# Autodesk Inventor assembly: BaseAssemblies
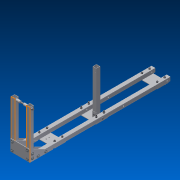
[picture p0: Inventor's stored thumbnail of the model, 180x180]
Saved by Autodesk Inventor 2013 (Build 170138000, 138)
## iProperties
Created: 2013-07-13
Part Number: BaseAssemblies
Document SubType Name: Assembly
Designer: orange
Mass: 2338.35 g
Surface Area: 7297.78 cm^2
Volume: 712.492 cm^3
Density: 3.28194 g/cm^3
Author: orange
## Documents named in this file (22)
- I:\FRC_Projects\Cad\Inventor_Projects\Shooter-Cleaned\BaseAssembly\BaseAssemblies.iam
- I:\FRC_Projects\Cad\Inventor_Projects\Shooter-Cleaned\BaseAssembly\Front_Bar.ipt
- I:\FRC_Projects\Cad\Inventor_Projects\Shooter-Cleaned\BaseAssembly\Support_Front.ipt
- I:\FRC_Projects\Cad\Inventor_Projects\Shooter-Cleaned\BaseAssembly\Support_Side_Front.ipt
- I:\FRC_Projects\Cad\Inventor_Projects\Shooter-Cleaned\Libraries\KOP\DBK_14-20x175_SHCS_am-1058.ipt
- I:\FRC_Projects\Cad\Inventor_Projects\Shooter-Cleaned\Libraries\KOP\DBK_14Washer_am-1027.ipt
- I:\FRC_Projects\Cad\Inventor_Projects\Shooter-Cleaned\Libraries\KOP\DBK_Nylock_14_20_am-1015.ipt
- I:\FRC_Projects\Cad\Inventor_Projects\Shooter-Cleaned\BaseAssembly\Bottom_Bar.ipt
- I:\FRC_Projects\Cad\Inventor_Projects\Shooter-Cleaned\BaseAssembly\Bolt_With_Washer.iam
- I:\FRC_Projects\Cad\Inventor_Projects\Shooter-Cleaned\Libraries\ContentCenter\ANSI_ASME B18.2.1 - 3_8-16 UNC - 5.5(2).ipt
- I:\FRC_Projects\Cad\Inventor_Projects\Shooter-Cleaned\Libraries\ContentCenter\ANSI B18.2.2 - 3_8 - 16(2).ipt
- I:\FRC_Projects\Cad\Inventor_Projects\Shooter-Cleaned\BaseAssembly\Spacer.ipt
- I:\FRC_Projects\Cad\Inventor_Projects\Shooter-Cleaned\BaseAssembly\CylinderPlate.ipt
- I:\FRC_Projects\Cad\Inventor_Projects\Shooter-Cleaned\Libraries\ContentCenter\ANSI B18.2.2 - 1_4 - 20(2).ipt
- I:\FRC_Projects\Cad\Inventor_Projects\Shooter-Cleaned\Libraries\ContentCenter\ANSI_ASME B18.2.1 - 1_4-20 UNC - 1.5(2).ipt
- I:\FRC_Projects\Cad\Inventor_Projects\Shooter-Cleaned\BaseAssembly\MountSwitchBar.ipt
- I:\FRC_Projects\Cad\Inventor_Projects\Shooter-Cleaned\BaseAssembly\SwitchBarSupport.ipt
- I:\FRC_Projects\Cad\Inventor_Projects\Shooter-Cleaned\BaseAssembly\LBrace.ipt
- I:\FRC_Projects\Cad\Inventor_Projects\Shooter-Cleaned\Libraries\ContentCenter\ANSI_ASME B18.2.1 - 1_4-20 UNC - 0.5(2).ipt
- I:\FRC_Projects\Cad\Inventor_Projects\Shooter-Cleaned\Libraries\ContentCenter\ANSI_ASME B18.2.1 - 1_4-20 UNC - 1.75(2).ipt
- I:\FRC_Projects\Cad\Inventor_Projects\Shooter-Cleaned\Libraries\ContentCenter\ANSI_ASME B18.2.1 - 1_4-20 UNC - 2.25(2).ipt
- I:\FRC_Projects\Cad\Inventor_Projects\Shooter-Cleaned\BaseAssembly\BackSuportPlate.ipt
## Components (80 placed, 21 different names)
1. Front_Bar:1 — Mate:1, Flush:2, Flush:3, Flush:5, Flush:6, Mate:3, Mate:6, Mate:17, Mate:19, Mate:32, Flush:7, Mate:79, Mate:83
2. Support_Front:1 — Mate:1, Flush:2, Flush:3, Mate:7, Mate:10, Mate:11, Mate:14, Mate:15, Mate:44, Mate:45, Mate:46, Mate:47, Mate:50, Mate:56
3. Support_Side_Front:1 — Mate:6, Mate:7, Mate:29, Mate:31, Mate:41, Mate:43
4. Support_Side_Front:2 — Flush:5, Flush:6, Mate:3, Mate:22, Mate:23, Mate:26, Mate:27, Mate:33, Mate:36, Mate:37, Mate:38, Mate:39
5. DBK_14-20x175_SHCS_am-1058:1 — Mate:8, Mate:9, Mate:10, Mate:16
6. DBK_14Washer_am-1027:1 — Mate:8, Mate:9, Mate:11
7. DBK_14-20x175_SHCS_am-1058:2 — Mate:12, Mate:13, Mate:14, Mate:18
8. DBK_14Washer_am-1027:2 — Mate:12, Mate:13, Mate:15
9. DBK_Nylock_14_20_am-1015:1 — Mate:16, Mate:17
10. DBK_Nylock_14_20_am-1015:2 — Mate:18, Mate:19
11. DBK_14Washer_am-1027:3 — Mate:20, Mate:21, Mate:22
12. DBK_14-20x175_SHCS_am-1058:3 — Mate:20, Mate:21, Mate:23, Mate:28
13. DBK_14-20x175_SHCS_am-1058:4 — Mate:24, Mate:25, Mate:27, Mate:30
14. DBK_14Washer_am-1027:4 — Mate:24, Mate:25, Mate:26
15. DBK_Nylock_14_20_am-1015:3 — Mate:28, Mate:29
16. DBK_Nylock_14_20_am-1015:4 — Mate:30, Mate:31
17. Bottom_Bar:1 — Mate:32, Mate:33, Flush:7, Mate:86, Flush:12, Mate:87, Mate:88, Mate:89, Mate:96, Mate:98, Mate:105, Flush:13, Mate:108, Mate:110, Mate:134, Mate:136, Mate:145, Mate:146, Mate:149, Mate:150, Mate:153, Mate:154, Mate:156, Mate:157, Mate:159
18. DBK_14-20x175_SHCS_am-1058:5 — Mate:34, Mate:35, Mate:36, Mate:42
19. DBK_14Washer_am-1027:5 — Mate:34, Mate:35, Mate:37
20. Bolt_With_Washer:1 [sub-assembly] — Mate:38, Mate:39, Mate:40
21. DBK_Nylock_14_20_am-1015:5 — Mate:40, Mate:41
22. DBK_Nylock_14_20_am-1015:6 — Mate:42, Mate:43
23. Front_Bar:2 — Mate:48, Mate:49, Mate:50, Mate:53, Mate:54, Mate:55, Flush:8, Flush:9, Flush:10, Mate:76, Mate:77, Mate:81
24. Bolt_With_Washer:2 [sub-assembly] — Mate:44, Mate:47, Mate:48, Mate:51
25. Bolt_With_Washer:3 [sub-assembly] — Mate:45, Mate:46, Mate:49, Mate:52
26. DBK_Nylock_14_20_am-1015:7 — Mate:51, Mate:53
27. DBK_Nylock_14_20_am-1015:8 — Mate:52, Mate:54
28. Support_Side_Front:3 — Mate:56, Flush:10, Mate:63, Mate:64, Mate:65, Mate:66, Mate:67, Mate:74, Mate:75
29. Support_Side_Front:4 — Mate:55, Flush:8, Flush:9, Mate:57, Mate:58, Mate:59, Mate:60, Mate:70, Mate:71, Mate:84
30. Bolt_With_Washer:4 [sub-assembly] — Mate:57, Mate:60, Mate:61
31. Bolt_With_Washer:5 [sub-assembly] — Mate:58, Mate:59, Mate:62
32. DBK_Nylock_14_20_am-1015:9 — Mate:61, Mate:63
33. DBK_Nylock_14_20_am-1015:10 — Mate:62, Mate:64
34. Bottom_Bar:2 — Mate:65, Mate:66, Mate:67, Mate:68, Mate:69, Mate:84, Mate:85, Flush:11, Mate:93, Mate:94, Mate:101, Mate:102, Mate:107, Mate:109, Mate:139, Mate:140, Mate:151, Mate:152, Mate:160, Mate:162, Mate:163, Mate:165
35. Bolt_With_Washer:6 [sub-assembly] — Mate:69, Mate:71, Mate:72
36. Bolt_With_Washer:7 [sub-assembly] — Mate:68, Mate:70, Mate:73
37. DBK_Nylock_14_20_am-1015:11 — Mate:73, Mate:75
38. DBK_Nylock_14_20_am-1015:12 — Mate:72, Mate:74
39. Hex Bolt - Inch 3/8-16 UNC - 5.5:1 — Mate:76, Mate:77, Mate:78, Mate:80, Mate:82
40. Hex Nut - Inch 3/8 - 16:1 — Mate:78, Mate:79
41. Spacer:1 — Mate:80, Mate:81
42. Spacer:2 — Mate:82, Mate:83
43. CylinderPlate:1 — Mate:85, Flush:11, Mate:86, Flush:12, Mate:87, Mate:88, Mate:90, Mate:91, Mate:92, Mate:103, Mate:104, Mate:106
44. Hex Nut - Inch 1/4 - 20:1 — Mate:95, Mate:96
45. Hex Nut - Inch 1/4 - 20:2 — Mate:97, Mate:98
46. Hex Nut - Inch 1/4 - 20:3 — Mate:100, Mate:101
47. Hex Nut - Inch 1/4 - 20:4 — Mate:99, Mate:102
48. Hex Bolt - Inch 1/4-20 UNC - 1.5:1 — Mate:89, Mate:90, Mate:97
49. Hex Bolt - Inch 1/4-20 UNC - 1.5:2 — Mate:91, Mate:92, Mate:95
50. Hex Bolt - Inch 1/4-20 UNC - 1.5:3 — Mate:93, Mate:99, Mate:104
51. Hex Bolt - Inch 1/4-20 UNC - 1.5:4 — Mate:94, Mate:100, Mate:103
52. MountSwitchBar:1 — Mate:105, Flush:13, Mate:106, Flush:14, Flush:15, Mate:108, Mate:109, Mate:113, Mate:116, Mate:117, Mate:118, Mate:119, Mate:120, Mate:125, Mate:126, Mate:127, Mate:128, Mate:129, Mate:130, Mate:131, Mate:132
53. SwitchBarSupport:1 — Flush:14, Mate:107, Flush:15, Mate:110, Mate:111, Mate:112, Mate:114, Mate:115, Mate:148
54. LBrace:1 — Mate:111, Mate:112, Mate:113, Mate:122, Mate:141, Mate:144
55. LBrace:2 — Mate:114, Mate:115, Mate:116, Mate:124, Mate:142
56. Hex Bolt - Inch 1/4-20 UNC - 0.5:1 — Mate:118, Mate:119, Mate:123
57. Hex Bolt - Inch 1/4-20 UNC - 0.5:2 — Mate:117, Mate:120, Mate:121
58. Hex Nut - Inch 1/4 - 20:5 — Mate:123, Mate:124
59. Hex Nut - Inch 1/4 - 20:6 — Mate:121, Mate:122
60. Hex Bolt - Inch 1/4-20 UNC - 1.75:1 — Mate:125, Mate:126, Mate:137
61. Hex Bolt - Inch 1/4-20 UNC - 1.75:2 — Mate:129, Mate:131, Mate:135
62. Hex Bolt - Inch 1/4-20 UNC - 1.75:3 — Mate:128, Mate:132, Mate:138
63. Hex Bolt - Inch 1/4-20 UNC - 1.75:4 — Mate:127, Mate:130, Mate:133
64. Hex Nut - Inch 1/4 - 20:7 — Mate:133, Mate:134
65. Hex Nut - Inch 1/4 - 20:8 — Mate:137, Mate:140
66. Hex Nut - Inch 1/4 - 20:9 — Mate:135, Mate:136
67. Hex Nut - Inch 1/4 - 20:10 — Mate:138, Mate:139
68. Hex Bolt - Inch 1/4-20 UNC - 1.5:5 — Mate:141, Mate:142, Mate:143
69. Hex Nut - Inch 1/4 - 20:11 — Mate:143, Mate:144
70. Hex Bolt - Inch 1/4-20 UNC - 2.25:1 — Mate:145, Mate:146, Mate:147
71. Hex Nut - Inch 1/4 - 20:12 — Mate:147, Mate:148
72. BackSuportPlate:1 — Mate:149, Mate:150, Mate:151, Mate:152, Mate:153, Mate:166, Mate:167, Mate:168, Mate:169
73. Hex Bolt - Inch 1/4-20 UNC - 1.5:6 — Mate:160, Mate:161, Mate:167
74. Hex Nut - Inch 1/4 - 20:13 — Mate:161, Mate:162
75. Hex Bolt - Inch 1/4-20 UNC - 1.5:7 — Mate:163, Mate:164, Mate:169
76. Hex Nut - Inch 1/4 - 20:14 — Mate:164, Mate:165
77. Hex Bolt - Inch 1/4-20 UNC - 1.5:8 — Mate:157, Mate:158, Mate:166
78. Hex Nut - Inch 1/4 - 20:15 — Mate:158, Mate:159
79. Hex Bolt - Inch 1/4-20 UNC - 1.5:9 — Mate:154, Mate:155, Mate:168
80. Hex Nut - Inch 1/4 - 20:16 — Mate:155, Mate:156
## Relationships (179: Mate 166, Flush 13)
- Mate:1: Front_Bar:1 ↔ Support_Front:1
- Flush:2: Front_Bar:1 ↔ Support_Front:1
- Flush:3: Front_Bar:1 ↔ Support_Front:1
- Flush:5: Front_Bar:1 ↔ Support_Side_Front:2
- Flush:6: Front_Bar:1 ↔ Support_Side_Front:2
- Mate:3: Front_Bar:1 ↔ Support_Side_Front:2
- Mate:6: Front_Bar:1 ↔ Support_Side_Front:1
- Mate:7: Support_Front:1 ↔ Support_Side_Front:1
- Mate:8: DBK_14-20x175_SHCS_am-1058:1 ↔ DBK_14Washer_am-1027:1
- Mate:9: DBK_14-20x175_SHCS_am-1058:1 ↔ DBK_14Washer_am-1027:1
- Mate:10: Support_Front:1 ↔ DBK_14-20x175_SHCS_am-1058:1
- Mate:11: Support_Front:1 ↔ DBK_14Washer_am-1027:1
- Mate:12: DBK_14-20x175_SHCS_am-1058:2 ↔ DBK_14Washer_am-1027:2
- Mate:13: DBK_14-20x175_SHCS_am-1058:2 ↔ DBK_14Washer_am-1027:2
- Mate:14: Support_Front:1 ↔ DBK_14-20x175_SHCS_am-1058:2
- Mate:15: Support_Front:1 ↔ DBK_14Washer_am-1027:2
- Mate:16: DBK_14-20x175_SHCS_am-1058:1 ↔ DBK_Nylock_14_20_am-1015:1
- Mate:17: Front_Bar:1 ↔ DBK_Nylock_14_20_am-1015:1
- Mate:18: DBK_14-20x175_SHCS_am-1058:2 ↔ DBK_Nylock_14_20_am-1015:2
- Mate:19: Front_Bar:1 ↔ DBK_Nylock_14_20_am-1015:2
- Mate:20: DBK_14Washer_am-1027:3 ↔ DBK_14-20x175_SHCS_am-1058:3
- Mate:21: DBK_14Washer_am-1027:3 ↔ DBK_14-20x175_SHCS_am-1058:3
- Mate:22: Support_Side_Front:2 ↔ DBK_14Washer_am-1027:3
- Mate:23: Support_Side_Front:2 ↔ DBK_14-20x175_SHCS_am-1058:3
- Mate:24: DBK_14-20x175_SHCS_am-1058:4 ↔ DBK_14Washer_am-1027:4
- Mate:25: DBK_14-20x175_SHCS_am-1058:4 ↔ DBK_14Washer_am-1027:4
- Mate:26: Support_Side_Front:2 ↔ DBK_14Washer_am-1027:4
- Mate:27: Support_Side_Front:2 ↔ DBK_14-20x175_SHCS_am-1058:4
- Mate:28: DBK_14-20x175_SHCS_am-1058:3 ↔ DBK_Nylock_14_20_am-1015:3
- Mate:29: Support_Side_Front:1 ↔ DBK_Nylock_14_20_am-1015:3
- Mate:30: DBK_14-20x175_SHCS_am-1058:4 ↔ DBK_Nylock_14_20_am-1015:4
- Mate:31: Support_Side_Front:1 ↔ DBK_Nylock_14_20_am-1015:4
- Mate:32: Front_Bar:1 ↔ Bottom_Bar:1
- Mate:33: Support_Side_Front:2 ↔ Bottom_Bar:1
- Flush:7: Front_Bar:1 ↔ Bottom_Bar:1
- Mate:34: DBK_14-20x175_SHCS_am-1058:5 ↔ DBK_14Washer_am-1027:5
- Mate:35: DBK_14-20x175_SHCS_am-1058:5 ↔ DBK_14Washer_am-1027:5
- Mate:36: Support_Side_Front:2 ↔ DBK_14-20x175_SHCS_am-1058:5
- Mate:37: Support_Side_Front:2 ↔ DBK_14Washer_am-1027:5
- Mate:38: Support_Side_Front:2 ↔ Bolt_With_Washer:1
- Mate:39: Support_Side_Front:2 ↔ Bolt_With_Washer:1
- Mate:40: Bolt_With_Washer:1 ↔ DBK_Nylock_14_20_am-1015:5
- Mate:41: Support_Side_Front:1 ↔ DBK_Nylock_14_20_am-1015:5
- Mate:42: DBK_14-20x175_SHCS_am-1058:5 ↔ DBK_Nylock_14_20_am-1015:6
- Mate:43: Support_Side_Front:1 ↔ DBK_Nylock_14_20_am-1015:6
- Mate:44: Support_Front:1 ↔ Bolt_With_Washer:2
- Mate:45: Support_Front:1 ↔ Bolt_With_Washer:3
- Mate:46: Support_Front:1 ↔ Bolt_With_Washer:3
- Mate:47: Support_Front:1 ↔ Bolt_With_Washer:2
- Mate:48: Front_Bar:2 ↔ Bolt_With_Washer:2
- Mate:49: Front_Bar:2 ↔ Bolt_With_Washer:3
- Mate:50: Support_Front:1 ↔ Front_Bar:2
- Mate:51: Bolt_With_Washer:2 ↔ DBK_Nylock_14_20_am-1015:7
- Mate:52: Bolt_With_Washer:3 ↔ DBK_Nylock_14_20_am-1015:8
- Mate:53: Front_Bar:2 ↔ DBK_Nylock_14_20_am-1015:7
- Mate:54: Front_Bar:2 ↔ DBK_Nylock_14_20_am-1015:8
- Mate:55: Front_Bar:2 ↔ Support_Side_Front:4
- Flush:8: Front_Bar:2 ↔ Support_Side_Front:4
- Flush:9: Front_Bar:2 ↔ Support_Side_Front:4
- Mate:56: Support_Front:1 ↔ Support_Side_Front:3
- Flush:10: Front_Bar:2 ↔ Support_Side_Front:3
- Mate:57: Support_Side_Front:4 ↔ Bolt_With_Washer:4
- Mate:58: Support_Side_Front:4 ↔ Bolt_With_Washer:5
- Mate:59: Support_Side_Front:4 ↔ Bolt_With_Washer:5
- Mate:60: Support_Side_Front:4 ↔ Bolt_With_Washer:4
- Mate:61: Bolt_With_Washer:4 ↔ DBK_Nylock_14_20_am-1015:9
- Mate:62: Bolt_With_Washer:5 ↔ DBK_Nylock_14_20_am-1015:10
- Mate:63: Support_Side_Front:3 ↔ DBK_Nylock_14_20_am-1015:9
- Mate:64: Support_Side_Front:3 ↔ DBK_Nylock_14_20_am-1015:10
- Mate:65: Support_Side_Front:3 ↔ Bottom_Bar:2
- Mate:66: Support_Side_Front:3 ↔ Bottom_Bar:2
- Mate:67: Support_Side_Front:3 ↔ Bottom_Bar:2
- Mate:68: Bottom_Bar:2 ↔ Bolt_With_Washer:7
- Mate:69: Bottom_Bar:2 ↔ Bolt_With_Washer:6
- Mate:70: Support_Side_Front:4 ↔ Bolt_With_Washer:7
- Mate:71: Support_Side_Front:4 ↔ Bolt_With_Washer:6
- Mate:72: Bolt_With_Washer:6 ↔ DBK_Nylock_14_20_am-1015:12
- Mate:73: Bolt_With_Washer:7 ↔ DBK_Nylock_14_20_am-1015:11
- Mate:74: Support_Side_Front:3 ↔ DBK_Nylock_14_20_am-1015:12
- Mate:75: Support_Side_Front:3 ↔ DBK_Nylock_14_20_am-1015:11
- Mate:76: Front_Bar:2 ↔ Hex Bolt - Inch 3/8-16 UNC - 5.5:1
- Mate:77: Front_Bar:2 ↔ Hex Bolt - Inch 3/8-16 UNC - 5.5:1
- Mate:78: Hex Bolt - Inch 3/8-16 UNC - 5.5:1 ↔ Hex Nut - Inch 3/8 - 16:1
- Mate:79: Front_Bar:1 ↔ Hex Nut - Inch 3/8 - 16:1
- Mate:80: Hex Bolt - Inch 3/8-16 UNC - 5.5:1 ↔ Spacer:1
- Mate:81: Front_Bar:2 ↔ Spacer:1
- Mate:82: Hex Bolt - Inch 3/8-16 UNC - 5.5:1 ↔ Spacer:2
- Mate:83: Front_Bar:1 ↔ Spacer:2
- Mate:84: Support_Side_Front:4 ↔ Bottom_Bar:2
- Mate:85: Bottom_Bar:2 ↔ CylinderPlate:1
- Flush:11: Bottom_Bar:2 ↔ CylinderPlate:1
- Mate:86: Bottom_Bar:1 ↔ CylinderPlate:1
- Flush:12: Bottom_Bar:1 ↔ CylinderPlate:1
- Mate:87: Bottom_Bar:1 ↔ CylinderPlate:1
- Mate:88: Bottom_Bar:1 ↔ CylinderPlate:1
- Mate:89: Bottom_Bar:1 ↔ Hex Bolt - Inch 1/4-20 UNC - 1.5:1
- Mate:90: CylinderPlate:1 ↔ Hex Bolt - Inch 1/4-20 UNC - 1.5:1
- Mate:91: CylinderPlate:1 ↔ Hex Bolt - Inch 1/4-20 UNC - 1.5:2
- Mate:92: CylinderPlate:1 ↔ Hex Bolt - Inch 1/4-20 UNC - 1.5:2
- Mate:93: Bottom_Bar:2 ↔ Hex Bolt - Inch 1/4-20 UNC - 1.5:3
- Mate:94: Bottom_Bar:2 ↔ Hex Bolt - Inch 1/4-20 UNC - 1.5:4
- Mate:95: Hex Nut - Inch 1/4 - 20:1 ↔ Hex Bolt - Inch 1/4-20 UNC - 1.5:2
- Mate:96: Bottom_Bar:1 ↔ Hex Nut - Inch 1/4 - 20:1
- Mate:97: Hex Nut - Inch 1/4 - 20:2 ↔ Hex Bolt - Inch 1/4-20 UNC - 1.5:1
- Mate:98: Bottom_Bar:1 ↔ Hex Nut - Inch 1/4 - 20:2
- Mate:99: Hex Nut - Inch 1/4 - 20:4 ↔ Hex Bolt - Inch 1/4-20 UNC - 1.5:3
- Mate:100: Hex Nut - Inch 1/4 - 20:3 ↔ Hex Bolt - Inch 1/4-20 UNC - 1.5:4
- Mate:101: Bottom_Bar:2 ↔ Hex Nut - Inch 1/4 - 20:3
- Mate:102: Bottom_Bar:2 ↔ Hex Nut - Inch 1/4 - 20:4
- Mate:103: CylinderPlate:1 ↔ Hex Bolt - Inch 1/4-20 UNC - 1.5:4
- Mate:104: CylinderPlate:1 ↔ Hex Bolt - Inch 1/4-20 UNC - 1.5:3
- Mate:105: Bottom_Bar:1 ↔ MountSwitchBar:1
- Flush:13: Bottom_Bar:1 ↔ MountSwitchBar:1
- Mate:106 (203.2 mm): CylinderPlate:1 ↔ MountSwitchBar:1
- Flush:14: MountSwitchBar:1 ↔ SwitchBarSupport:1
- Mate:107 (50.8 mm): Bottom_Bar:2 ↔ SwitchBarSupport:1
- Flush:15 (-25.4 mm): MountSwitchBar:1 ↔ SwitchBarSupport:1
- Mate:108: Bottom_Bar:1 ↔ MountSwitchBar:1
- Mate:109: Bottom_Bar:2 ↔ MountSwitchBar:1
- Mate:110: Bottom_Bar:1 ↔ SwitchBarSupport:1
- Mate:111: SwitchBarSupport:1 ↔ LBrace:1
- Mate:112: SwitchBarSupport:1 ↔ LBrace:1
- Mate:113: MountSwitchBar:1 ↔ LBrace:1
- Mate:114: SwitchBarSupport:1 ↔ LBrace:2
- Mate:115: SwitchBarSupport:1 ↔ LBrace:2
- Mate:116: MountSwitchBar:1 ↔ LBrace:2
- Mate:117: MountSwitchBar:1 ↔ Hex Bolt - Inch 1/4-20 UNC - 0.5:2
- Mate:118: MountSwitchBar:1 ↔ Hex Bolt - Inch 1/4-20 UNC - 0.5:1
- Mate:119: MountSwitchBar:1 ↔ Hex Bolt - Inch 1/4-20 UNC - 0.5:1
- Mate:120: MountSwitchBar:1 ↔ Hex Bolt - Inch 1/4-20 UNC - 0.5:2
- Mate:121: Hex Bolt - Inch 1/4-20 UNC - 0.5:2 ↔ Hex Nut - Inch 1/4 - 20:6
- Mate:122: LBrace:1 ↔ Hex Nut - Inch 1/4 - 20:6
- Mate:123: Hex Bolt - Inch 1/4-20 UNC - 0.5:1 ↔ Hex Nut - Inch 1/4 - 20:5
- Mate:124: LBrace:2 ↔ Hex Nut - Inch 1/4 - 20:5
- Mate:125: MountSwitchBar:1 ↔ Hex Bolt - Inch 1/4-20 UNC - 1.75:1
- Mate:126: MountSwitchBar:1 ↔ Hex Bolt - Inch 1/4-20 UNC - 1.75:1
- Mate:127: MountSwitchBar:1 ↔ Hex Bolt - Inch 1/4-20 UNC - 1.75:4
- Mate:128: MountSwitchBar:1 ↔ Hex Bolt - Inch 1/4-20 UNC - 1.75:3
- Mate:129: MountSwitchBar:1 ↔ Hex Bolt - Inch 1/4-20 UNC - 1.75:2
- Mate:130: MountSwitchBar:1 ↔ Hex Bolt - Inch 1/4-20 UNC - 1.75:4
- Mate:131: MountSwitchBar:1 ↔ Hex Bolt - Inch 1/4-20 UNC - 1.75:2
- Mate:132: MountSwitchBar:1 ↔ Hex Bolt - Inch 1/4-20 UNC - 1.75:3
- Mate:133: Hex Bolt - Inch 1/4-20 UNC - 1.75:4 ↔ Hex Nut - Inch 1/4 - 20:7
- Mate:134: Bottom_Bar:1 ↔ Hex Nut - Inch 1/4 - 20:7
- Mate:135: Hex Bolt - Inch 1/4-20 UNC - 1.75:2 ↔ Hex Nut - Inch 1/4 - 20:9
- Mate:136: Bottom_Bar:1 ↔ Hex Nut - Inch 1/4 - 20:9
- Mate:137: Hex Bolt - Inch 1/4-20 UNC - 1.75:1 ↔ Hex Nut - Inch 1/4 - 20:8
- Mate:138: Hex Bolt - Inch 1/4-20 UNC - 1.75:3 ↔ Hex Nut - Inch 1/4 - 20:10
- Mate:139: Bottom_Bar:2 ↔ Hex Nut - Inch 1/4 - 20:10
- Mate:140: Bottom_Bar:2 ↔ Hex Nut - Inch 1/4 - 20:8
- Mate:141: LBrace:1 ↔ Hex Bolt - Inch 1/4-20 UNC - 1.5:5
- Mate:142: LBrace:2 ↔ Hex Bolt - Inch 1/4-20 UNC - 1.5:5
- Mate:143: Hex Bolt - Inch 1/4-20 UNC - 1.5:5 ↔ Hex Nut - Inch 1/4 - 20:11
- Mate:144: LBrace:1 ↔ Hex Nut - Inch 1/4 - 20:11
- Mate:145: Bottom_Bar:1 ↔ Hex Bolt - Inch 1/4-20 UNC - 2.25:1
- Mate:146: Bottom_Bar:1 ↔ Hex Bolt - Inch 1/4-20 UNC - 2.25:1
- Mate:147: Hex Bolt - Inch 1/4-20 UNC - 2.25:1 ↔ Hex Nut - Inch 1/4 - 20:12
- Mate:148: SwitchBarSupport:1 ↔ Hex Nut - Inch 1/4 - 20:12
- Mate:149: Bottom_Bar:1 ↔ BackSuportPlate:1
- Mate:150: Bottom_Bar:1 ↔ BackSuportPlate:1
- Mate:151: Bottom_Bar:2 ↔ BackSuportPlate:1
- Mate:152: Bottom_Bar:2 ↔ BackSuportPlate:1
- Mate:153: Bottom_Bar:1 ↔ BackSuportPlate:1
- Mate:154: Bottom_Bar:1 ↔ Hex Bolt - Inch 1/4-20 UNC - 1.5:9
- Mate:155: Hex Bolt - Inch 1/4-20 UNC - 1.5:9 ↔ Hex Nut - Inch 1/4 - 20:16
- Mate:156: Bottom_Bar:1 ↔ Hex Nut - Inch 1/4 - 20:16
- Mate:157: Bottom_Bar:1 ↔ Hex Bolt - Inch 1/4-20 UNC - 1.5:8
- Mate:158: Hex Bolt - Inch 1/4-20 UNC - 1.5:8 ↔ Hex Nut - Inch 1/4 - 20:15
- Mate:159: Bottom_Bar:1 ↔ Hex Nut - Inch 1/4 - 20:15
- Mate:160: Bottom_Bar:2 ↔ Hex Bolt - Inch 1/4-20 UNC - 1.5:6
- Mate:161: Hex Bolt - Inch 1/4-20 UNC - 1.5:6 ↔ Hex Nut - Inch 1/4 - 20:13
- Mate:162: Bottom_Bar:2 ↔ Hex Nut - Inch 1/4 - 20:13
- Mate:163: Bottom_Bar:2 ↔ Hex Bolt - Inch 1/4-20 UNC - 1.5:7
- Mate:164: Hex Bolt - Inch 1/4-20 UNC - 1.5:7 ↔ Hex Nut - Inch 1/4 - 20:14
- Mate:165: Bottom_Bar:2 ↔ Hex Nut - Inch 1/4 - 20:14
- Mate:166: BackSuportPlate:1 ↔ Hex Bolt - Inch 1/4-20 UNC - 1.5:8
- Mate:167: BackSuportPlate:1 ↔ Hex Bolt - Inch 1/4-20 UNC - 1.5:6
- Mate:168: BackSuportPlate:1 ↔ Hex Bolt - Inch 1/4-20 UNC - 1.5:9
- Mate:169: BackSuportPlate:1 ↔ Hex Bolt - Inch 1/4-20 UNC - 1.5:7
